# Autodesk Inventor assembly: ASY MSC 002 отстойник осветлитель
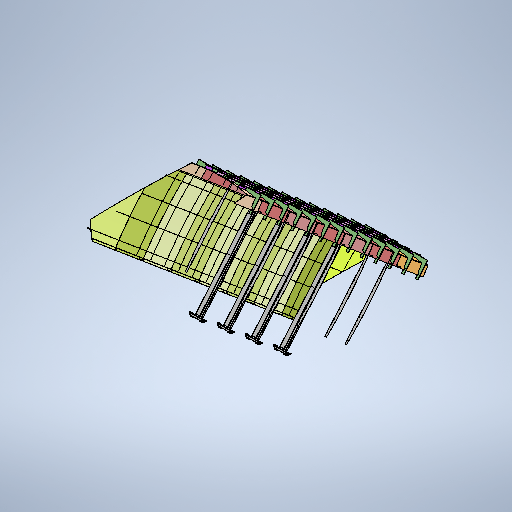
[picture p0: Inventor's stored thumbnail of the model, 512x512]
Saved by Autodesk Inventor 2025.1 (Build 291241020, 241B)
## iProperties
allow_slope_adjustment: 0 ul
flow_configuration: 1 ul
flow_direction: 2 ul
loss_method: 0 ul
radius: 110.000 mm
flow_configuration2: 1 ul
radius: 61.000 mm
radius: 44.450 mm
radius: 59.000 mm
Created: 2024-09-05
Part Number: ASY MSC 002 отстойник осветлитель
Document SubType Name: Assembly
Designer: admin
Mass: 3.32073e+06 g
Surface Area: 6.08214e+06 cm^2
Volume: 433030 cm^3
Density: 7.66859 g/cm^3
Author: admin
## Documents named in this file (52)
- C:\Users\user\YandexDisk-badmisterfox\домашниий пк\Inventor\Manturovo\Manturovo_Se-clar\ASY MSC 002 отстойник осветлитель.iam
- C:\Users\user\YandexDisk-badmisterfox\домашниий пк\Inventor\Manturovo\Manturovo_Se-clar\ASY MSC 900.1 base frame.iam
- C:\Users\user\YandexDisk-badmisterfox\домашниий пк\Inventor\Manturovo\Manturovo_Se-clar\ASY MSC 100 cone.iam
- C:\Users\user\YandexDisk-badmisterfox\домашниий пк\Inventor\Manturovo\Manturovo_Se-clar\MSC 401 sheet lowerback.ipt
- C:\Users\user\YandexDisk-badmisterfox\домашниий пк\Inventor\Manturovo\Manturovo_Se-clar\MSC 701 face 1.ipt
- C:\Users\user\YandexDisk-badmisterfox\домашниий пк\Inventor\Manturovo\Manturovo_Se-clar\MSC 705 ridge 3.ipt
- C:\Users\user\YandexDisk-badmisterfox\домашниий пк\Inventor\Manturovo\Manturovo_Se-clar\MSC 713 tube.ipt
- C:\Users\user\YandexDisk-badmisterfox\домашниий пк\Inventor\Manturovo\Manturovo_Se-clar\ISO 5251 Bends 3D without straight ends(90 deg) DN150 11 11.ipt
- C:\Users\user\YandexDisk-badmisterfox\домашниий пк\Inventor\Manturovo\Manturovo_Se-clar\MSC 408 stringer lowerback.ipt
- C:\Users\user\YandexDisk-badmisterfox\домашниий пк\Inventor\Manturovo\Manturovo_Se-clar\MSC 703 face 2.ipt
- C:\Users\user\YandexDisk-badmisterfox\домашниий пк\Inventor\Manturovo\Manturovo_Se-clar\MSC 702 face 3.ipt
- C:\Users\user\YandexDisk-badmisterfox\домашниий пк\Inventor\Manturovo\Manturovo_Se-clar\MSC 704 face 4.ipt
- C:\Users\user\YandexDisk-badmisterfox\домашниий пк\Inventor\Manturovo\Manturovo_Se-clar\ASY MSC 900.3 base frame.iam
- C:\Users\user\YandexDisk-badmisterfox\домашниий пк\Inventor\Manturovo\Manturovo_Se-clar\Pillars\ASY MSC 900.5 base frame.iam
- C:\Users\user\YandexDisk-badmisterfox\домашниий пк\Inventor\Manturovo\Manturovo_Se-clar\Pillars\ASY MSC 900.4  base frame.iam
- C:\Users\user\YandexDisk-badmisterfox\домашниий пк\Inventor\Manturovo\Manturovo_Se-clar\Pillars\ASY MSC 900.6 base frame.iam
- C:\Users\user\YandexDisk-badmisterfox\домашниий пк\Inventor\Manturovo\Manturovo_Se-clar\ASY MSC 200 BACK.iam
- C:\Users\user\YandexDisk-badmisterfox\домашниий пк\Inventor\Manturovo\Manturovo_Se-clar\ASY MSC 300.2 LEFT BOARD.iam
- C:\Users\user\YandexDisk-badmisterfox\домашниий пк\Inventor\Manturovo\Manturovo_Se-clar\ASY MSC 300.1 RIGHT BOARD.iam
- C:\Users\user\YandexDisk-badmisterfox\домашниий пк\Inventor\Manturovo\Manturovo_Se-clar\ASY MSC 500 BELLY.iam
- C:\Users\user\YandexDisk-badmisterfox\домашниий пк\Inventor\Manturovo\Manturovo_Se-clar\ASY MSC 900.2 support.iam
- C:\Users\user\YandexDisk-badmisterfox\домашниий пк\Inventor\Manturovo\Manturovo_Se-clar\ASY MSC 600 cone exit back.iam
- C:\Users\user\YandexDisk-badmisterfox\домашниий пк\Inventor\Manturovo\Manturovo_Se-clar\ASY MSC 800 gills.iam
- C:\Users\user\YandexDisk-badmisterfox\домашниий пк\Inventor\Manturovo\Manturovo_Se-clar\ASY MSC 400 Accsess hatch.iam
- C:\Users\user\YandexDisk-badmisterfox\домашниий пк\Inventor\Manturovo\Manturovo_Se-clar\MSC DIM 000 settler-clarifier.ipt
- C:\Users\user\YandexDisk-badmisterfox\домашниий пк\Inventor\Manturovo\Manturovo_Se-clar\MSC DIM 001 frame.ipt
- C:\Users\user\YandexDisk-badmisterfox\домашниий пк\Inventor\Manturovo\Manturovo_Se-clar\ASY MSC 900.7 base frame transverse.iam
- C:\Users\user\YandexDisk-badmisterfox\домашниий пк\Inventor\Manturovo\Manturovo_Se-clar\ASY MSC 900.8 base frame transverse.iam
- C:\Users\user\YandexDisk-badmisterfox\домашниий пк\Inventor\Manturovo\Manturovo_Se-clar\MSC 908 transverse pillar plate.ipt
- C:\Users\user\YandexDisk-badmisterfox\домашниий пк\Inventor\Manturovo\Manturovo_Se-clar\MSC 900.9 base frame transverse.ipt
- C:\Users\user\YandexDisk-badmisterfox\домашниий пк\Inventor\Manturovo\Manturovo_Se-clar\ASY MSC 700 water tray.iam
- C:\Users\user\YandexDisk-badmisterfox\домашниий пк\Inventor\Manturovo\Manturovo_Se-clar\ASY 940 linkage.iam
- C:\Users\user\YandexDisk-badmisterfox\домашниий пк\Inventor\Manturovo\Manturovo_Se-clar\MSC 510 BELLY PILLAR.ipt
- C:\Users\user\YandexDisk-badmisterfox\домашниий пк\Inventor\Manturovo\Manturovo_Se-clar\ASY MSC 900.7 support.iam
- C:\Users\user\YandexDisk-badmisterfox\домашниий пк\Inventor\Manturovo\Manturovo_Se-clar\Content Center Files\en-US\DIN 2605 90 T 3\DIN 2605 90 Deg Elbow Type 2 168.3 - 2.6S.ipt
- C:\Users\admin\YandexDisk-badmisterfox\домашниий пк\Inventor\Manturovo\Manturovo_Se-clar\3d party\Stamp flange DIN2642\Stamd flange lapped collar DIN2642.ipt
- C:\Users\user\YandexDisk-badmisterfox\домашниий пк\Inventor\Manturovo\Manturovo_Se-clar\3d party\Stamp flange DIN2642\Stamd flange lapped collar DIN2642\Stamp flange DIN2642-150.ipt
- C:\Users\user\YandexDisk-badmisterfox\домашниий пк\Inventor\Manturovo\Manturovo_Se-clar\Content Center Files\en-US\DIN 2605 90 T 3\DIN 2605 90 Deg Elbow Type 2 88.9 - 2.3S.ipt
- C:\Users\user\YandexDisk-badmisterfox\домашниий пк\Inventor\Manturovo\Manturovo_Se-clar\Stamp flange DIN2642-080.ipt
- C:\Users\user\YandexDisk-badmisterfox\домашниий пк\Inventor\Manturovo\Manturovo_Se-clar\DIN EN ISO 1127(1) - 88,9 x 2,3 - 100.ipt
- C:\Users\user\YandexDisk-badmisterfox\домашниий пк\Inventor\Manturovo\Manturovo_Se-clar\3d party\Stamp flange DIN2642\Stamd flange lapped collar DIN2642.ipt
- C:\Users\user\YandexDisk-badmisterfox\домашниий пк\Inventor\Manturovo\Manturovo_Se-clar\3d party\Butterfly value\butterfly-valve-3-in-1.snapshot.4\vpe_3449-02_dn80_.iam
- C:\Users\user\YandexDisk-badmisterfox\домашниий пк\Inventor\Manturovo\Manturovo_Se-clar\LASER\4 очередь\D-ring 11.ipt
- C:\Users\user\YandexDisk-badmisterfox\домашниий пк\Inventor\Manturovo\Manturovo_Se-clar\MSC 606 rocket tube 6.ipt
- C:\Users\user\YandexDisk-badmisterfox\домашниий пк\Inventor\Manturovo\Manturovo_Se-clar\Stamp flange DIN2642-065.ipt
- C:\Users\user\YandexDisk-badmisterfox\домашниий пк\Inventor\Manturovo\Manturovo_Se-clar\ContentCenter\en-US\ISO 5251 B 3D\ISO 5251 Bends 3D without straight ends(90 deg) DN65 2.9 2.9.ipt
- C:\Users\user\YandexDisk-badmisterfox\домашниий пк\Inventor\Manturovo\Manturovo_Se-clar\MSC 616 belly tube 16.ipt
- C:\Users\user\YandexDisk-badmisterfox\домашниий пк\Inventor\Manturovo\Manturovo_Se-clar\MSC 617 belly tube 17.ipt
- C:\Users\user\YandexDisk-badmisterfox\домашниий пк\Inventor\Manturovo\Manturovo_Se-clar\MSC 618 belly tube 18.ipt
- C:\Users\user\YandexDisk-badmisterfox\домашниий пк\Inventor\Manturovo\Manturovo_Se-clar\MSC 808 sheet.ipt
- C:\Users\user\YandexDisk-badmisterfox\домашниий пк\Inventor\Manturovo\Manturovo_Se-clar\DIN EN 10219-2 - 40 x 20 x 2  - 2000.ipt
- C:\Users\user\YandexDisk-badmisterfox\домашниий пк\Inventor\Manturovo\Manturovo_Se-clar\MSC 813 wall support gills.ipt
## Components (80 placed, 52 different names)
1. MSC DIM 000 settler-clarifier.ipt:1
2. MSC DIM 001 frame.ipt:1
3. ASY MSC 900.4  base frame.iam:1 [sub-assembly] — Mate:32, Mate:33, Mate:45, Mate:46, Cylindrical:11, Mate:82
4. ASY MSC 900.5 base frame.iam:1 [sub-assembly] — Flush:11, Cylindrical:7, Mate:46, Mate:48, Cylindrical:10
5. ASY MSC 900.6 base frame.iam:1 [sub-assembly] — Mate:38, Mate:39, Cylindrical:6, Mate:47, Rigid:19, Rigid:20, Rigid:21, Rigid:22, Cylindrical:9, Mate:84
6. ASY MSC 900.3 base frame.iam:1 [sub-assembly] — Mate:23, Mate:24, Mate:44, Mate:45, Rigid:31, Rigid:32, Rigid:33, Cylindrical:8
7. ASY MSC 900.8 base frame transverse.iam:1 [sub-assembly] — Rigid:22
8. ASY MSC 900.8 base frame transverse.iam:2 [sub-assembly] — Rigid:21
9. ASY MSC 900.7 base frame transverse.iam:1 [sub-assembly] — Rigid:19
10. ASY MSC 900.7 base frame transverse.iam:2 [sub-assembly] — Rigid:20
11. MSC 705 ridge 3.ipt:1
12. MSC 704 face 4.ipt:1
13. MSC 900.9 base frame transverse.ipt:4 — Mate:81, Mate:83
14. Part1:2 — Mate:81, Mate:82
15. Part1:4 — Mate:88
16. MSC 900.9 base frame transverse:7 — Mate:87, Mate:88
17. ASY MSC 900.2 support.iam:5 [sub-assembly]
18. ASY MSC 900.7 support:2 [sub-assembly] — Cylindrical:11, Mate:78
19. Part1:3 — Mate:84, Mate:85
20. MSC 900.9 base frame transverse.ipt:1 — Mate:85, Mate:86
21. MSC 900.9 base frame transverse.ipt:2
22. ASY MSC 900.2 support.iam:4 [sub-assembly] — Cylindrical:7, Mate:41
23. ASY MSC 900.7 support:3 [sub-assembly] — Cylindrical:10, Mate:79
24. MSC 701 face 1.ipt:1 — Rigid:4, Flush:9, Mate:35, Rigid:35, Rigid:36, Rigid:39, Rigid:40
25. ASY MSC 900.2 support.iam:1 [sub-assembly] — Cylindrical:6, Mate:42
26. MSC 702 face 3.ipt:1 — Mate:34, Mate:35, Mate:36, Mate:66
27. MSC 703 face 2.ipt:1 — Flush:13, Flush:17, Mate:66
28. MSC 713 tube.ipt:2
29. ISO 5251 Bends 3D without straight ends(90 deg) DN150 11 11.ipt:1
30. MSC 713 tube.ipt:1 — Rigid:4
31. ASY MSC 900.7 support:4 [sub-assembly] — Cylindrical:9, Mate:80
32. ASY MSC 700 water tray.iam:1 [sub-assembly]
33. Part1.ipt:1 — Rigid:33, Mate:68, Mate:69, Mate:70
34. MSC 900.9 base frame transverse.ipt:3 — Mate:68, Mate:69, Mate:70
35. ASY MSC 900.2 support.iam:8 [sub-assembly]
36. ASY MSC 900.7 support:1 [sub-assembly] — Cylindrical:8, Mate:77
37. ASY MSC 600 cone exit back.iam:1 [sub-assembly] — Rigid:17
38. MSC 908 transverse pillar plate.ipt:1
39. MSC 908 transverse pillar plate.ipt:2 — Mate:50, Flush:16, Flush:18
40. MSC 401 sheet lowerback.ipt:1 — Mate:29, Mate:30, Rigid:34
41. ASY MSC 400 Accsess hatch.iam:1 [sub-assembly] — Rigid:34
42. MSC 408 stringer lowerback.ipt:2
43. MSC 408 stringer lowerback.ipt:1
44. ASY MSC 100 cone.iam:1 [sub-assembly] — Mate:19, Flush:6, Mate:29, Rigid:17, Rigid:48, Rigid:53
45. ASY MSC 900.1 base frame.iam:1 [sub-assembly] — Flush:5, Mate:19, Mate:44, Mate:47, Mate:50, Flush:16
46. ASY 940 linkage.iam:1 [sub-assembly] — Rigid:32, Flush:18
47. ASY 940 linkage.iam:2 [sub-assembly] — Rigid:31
48. ASY MSC 500 BELLY.iam:1 [sub-assembly] — Flush:7, Mate:22, Rigid:10, Rigid:11, Mate:41, Mate:42, Mate:77, Mate:78, Mate:79, Mate:80, Mate:83, Mate:86, Mate:87
49. ASY MSC 200 BACK.iam:1 [sub-assembly] — Flush:8
50. ASY MSC 300.2 LEFT BOARD.iam:1 [sub-assembly] — Rigid:11, Mate:34, Rigid:49
51. ASY MSC 300.1 RIGHT BOARD.iam:1 [sub-assembly] — Rigid:10, Flush:17
52. ASY MSC 800 gills.iam:1 [sub-assembly] — Mate:22, Rigid:56
53. DIN 2605 90 Deg Elbow Type 2 168.3 - 2.6S:1 — Rigid:36, Rigid:38
54. DIN 2605 90 Deg Elbow Type 2 168.3 - 2.6S:2 — Rigid:35, Rigid:37
55. Stamp flange DIN2642-150:1 — Rigid:38
56. Stamp flange DIN2642-150:3 — Rigid:37
57. DIN 2605 90 Deg Elbow Type 2 88.9 - 2.3S:1 — Rigid:39, Rotational:2
58. Stamp flange DIN2642-080:4 — Rotational:2
59. DIN EN ISO 1127(1) - 88,9 x 2,3 - 100:1 — Rigid:40
60. vpe_3449-02_dn80_:1 [sub-assembly] — Rigid:48
61. D-ring 11:1 — Rigid:41, Rigid:49
62. D-ring 11:2 — Rigid:41
63. MSC 606 rocket tube 6.ipt:1 — Rotational:4
64. ISO 5251 Bends 3D without straight ends(90 deg) DN65 2.9:1 — Rigid:45, Rigid:47
65. Stamp flange DIN2642-065.ipt:1 — Rotational:3, Rotational:6
66. ISO 5251 Bends 3D without straight ends(90 deg) DN65 2.9:2 — Rotational:3, Rigid:46
67. MSC 616 belly tube 16:1 — Rigid:45, Rigid:46
68. Stamp flange DIN2642-065:6 — Rigid:47, Rotational:5
69. Stamp flange DIN2642-065:7 — Rotational:4, Rotational:5
70. Stamp flange DIN2642-065:8 — Rotational:6, Rotational:7
71. MSC 617 belly tube 17:1 — Rotational:7, Rigid:50
72. Stamp flange DIN2642-065:9 — Rigid:50, Rigid:55
73. MSC 618 belly tube 18:1 — Rigid:52, Rigid:51
74. Stamp flange DIN2642-065:10 — Rigid:53, Rigid:52
75. Stamp flange DIN2642-065:11 — Rigid:51, Rigid:54
76. vpe_3449-02_dn80_:2 [sub-assembly] — Rigid:54
77. vpe_3449-02_dn80_:3 [sub-assembly] — Rigid:55
78. MSC 808 sheet:1
79. DIN EN 10219-2 - 40 x 20 x 2  - 2000:1
80. MSC 813 wall support gills:1 — Rigid:56
## Relationships (111: Mate 47, WeldJoint 37, Flush 12, CylindricalJoint 8, RevoluteJoint 7)
- [Mate]: MSC 401 sheet lowerback.ipt:1 ↔ ASY MSC 100 cone.iam:1
- [WeldJoint]: ISO 5251 Bends 3D without straight ends(90 deg) DN150 11 11.ipt:1 ↔ MSC 713 tube.ipt:1
- [Mate]: MSC 408 stringer lowerback.ipt:1 ↔ ASY MSC 100 cone.iam:1
- [RevoluteJoint]: MSC 713 tube.ipt:2 ↔ ISO 5251 Bends 3D without straight ends(90 deg) DN150 11 11.ipt:1
- Rigid:4 [WeldJoint]: MSC 701 face 1.ipt:1 ↔ MSC 713 tube.ipt:1
- [Mate]: MSC 408 stringer lowerback.ipt:2 ↔ ASY MSC 100 cone.iam:1
- [Mate]: ASY MSC 600 cone exit back.iam:1 ↔ ASY MSC 500 BELLY.iam:1
- [WeldJoint]: MSC 705 ridge 3.ipt:1 ↔ ASY MSC 700 water tray.iam:1
- [WeldJoint]: MSC 705 ridge 3.ipt:1 ↔ ASY MSC 700 water tray.iam:1
- [Flush]: ASY MSC 600 cone exit back.iam:1 ↔ ASY MSC 500 BELLY.iam:1
- [Mate]: ASY MSC 500 BELLY.iam:1 ↔ ASY MSC 800 gills.iam:1
- [Mate]: MSC 701 face 1.ipt:1 ↔ ASY MSC 500 BELLY.iam:1
- [Mate] (3 mm): MSC 701 face 1.ipt:1 ↔ ASY MSC 500 BELLY.iam:1
- [Mate] (3 mm): ASY MSC 900.2 support.iam:5 ↔ ASY MSC 500 BELLY.iam:1
- [Mate] (3 mm): ASY MSC 900.2 support.iam:8 ↔ ASY MSC 500 BELLY.iam:1
- [CylindricalJoint]: ASY MSC 900.4  base frame.iam:1 ↔ ASY MSC 900.2 support.iam:5
- [Mate] (-2860 mm): ASY MSC 500 BELLY.iam:1 ↔ ASY MSC 200 BACK.iam:1
- [CylindricalJoint]: ASY MSC 900.3 base frame.iam:1 ↔ ASY MSC 900.2 support.iam:8
- [Flush]: ASY MSC 900.4  base frame.iam:1 ↔ ASY MSC 900.3 base frame.iam:1
- Flush:5: ASY MSC 900.1 base frame.iam:1
- Mate:19: ASY MSC 100 cone.iam:1 ↔ ASY MSC 900.1 base frame.iam:1
- Flush:6: ASY MSC 100 cone.iam:1
- Flush:7: ASY MSC 500 BELLY.iam:1
- Flush:8: ASY MSC 200 BACK.iam:1
- Mate:22: ASY MSC 500 BELLY.iam:1 ↔ ASY MSC 800 gills.iam:1
- Mate:23: ASY MSC 900.3 base frame.iam:1
- Mate:24: ASY MSC 900.3 base frame.iam:1
- Flush:9: MSC 701 face 1.ipt:1
- Mate:29: MSC 401 sheet lowerback.ipt:1 ↔ ASY MSC 100 cone.iam:1
- Mate:30: MSC 401 sheet lowerback.ipt:1
- Rigid:10 [WeldJoint] (-25 mm): ASY MSC 500 BELLY.iam:1 ↔ ASY MSC 300.1 RIGHT BOARD.iam:1
- Rigid:11 [WeldJoint] (-25 mm): ASY MSC 500 BELLY.iam:1 ↔ ASY MSC 300.2 LEFT BOARD.iam:1
- Flush:11: ASY MSC 900.5 base frame.iam:1
- Mate:32: ASY MSC 900.4  base frame.iam:1
- Mate:33: ASY MSC 900.4  base frame.iam:1
- Mate:34: MSC 702 face 3.ipt:1 ↔ ASY MSC 300.2 LEFT BOARD.iam:1
- Mate:35: MSC 701 face 1.ipt:1 ↔ MSC 702 face 3.ipt:1
- [WeldJoint]: MSC 705 ridge 3.ipt:1 ↔ ASY MSC 700 water tray.iam:1
- Mate:36: MSC 702 face 3.ipt:1
- Mate:38: ASY MSC 900.6 base frame.iam:1
- Mate:39: ASY MSC 900.6 base frame.iam:1
- Cylindrical:6: ASY MSC 900.6 base frame.iam:1 ↔ ASY MSC 900.2 support.iam:1
- Cylindrical:7: ASY MSC 900.5 base frame.iam:1 ↔ ASY MSC 900.2 support.iam:4
- Mate:41 (3 mm): ASY MSC 900.2 support.iam:4 ↔ ASY MSC 500 BELLY.iam:1
- Mate:42 (3 mm): ASY MSC 900.2 support.iam:1 ↔ ASY MSC 500 BELLY.iam:1
- Flush:13: MSC 703 face 2.ipt:1
- Mate:44 (820 mm): ASY MSC 900.3 base frame.iam:1 ↔ ASY MSC 900.1 base frame.iam:1
- Mate:45 (1430 mm): ASY MSC 900.4  base frame.iam:1 ↔ ASY MSC 900.3 base frame.iam:1
- Mate:46 (1430 mm): ASY MSC 900.4  base frame.iam:1 ↔ ASY MSC 900.5 base frame.iam:1
- Mate:47 (5300 mm): ASY MSC 900.6 base frame.iam:1 ↔ ASY MSC 900.1 base frame.iam:1
- Rigid:17 [WeldJoint]: ASY MSC 600 cone exit back.iam:1 ↔ ASY MSC 100 cone.iam:1
- Mate:48: ASY MSC 900.5 base frame.iam:1
- Rigid:19 [WeldJoint]: ASY MSC 900.6 base frame.iam:1 ↔ ASY MSC 900.7 base frame transverse.iam:1
- Rigid:20 [WeldJoint]: ASY MSC 900.6 base frame.iam:1 ↔ ASY MSC 900.7 base frame transverse.iam:2
- Rigid:21 [WeldJoint]: ASY MSC 900.6 base frame.iam:1 ↔ ASY MSC 900.8 base frame transverse.iam:2
- Rigid:22 [WeldJoint]: ASY MSC 900.6 base frame.iam:1 ↔ ASY MSC 900.8 base frame transverse.iam:1
- Mate:50: MSC 908 transverse pillar plate.ipt:2 ↔ ASY MSC 900.1 base frame.iam:1
- Flush:16 (-40 mm): MSC 908 transverse pillar plate.ipt:2 ↔ ASY MSC 900.1 base frame.iam:1
- Flush:17: MSC 703 face 2.ipt:1 ↔ ASY MSC 300.1 RIGHT BOARD.iam:1
- Mate:66: MSC 702 face 3.ipt:1 ↔ MSC 703 face 2.ipt:1
- [WeldJoint]: MSC 908 transverse pillar plate.ipt:1 ↔ ASY 940 linkage.iam:2
- Rigid:31 [WeldJoint]: ASY MSC 900.3 base frame.iam:1 ↔ ASY 940 linkage.iam:2
- Rigid:32 [WeldJoint]: ASY MSC 900.3 base frame.iam:1 ↔ ASY 940 linkage.iam:1
- Flush:18: MSC 908 transverse pillar plate.ipt:2 ↔ ASY 940 linkage.iam:1
- Rigid:33 [WeldJoint]: ASY MSC 900.3 base frame.iam:1 ↔ Part1.ipt:1
- Mate:68: Part1.ipt:1 ↔ MSC 900.9 base frame transverse.ipt:3
- Mate:69 (11 mm): Part1.ipt:1 ↔ MSC 900.9 base frame transverse.ipt:3
- Mate:70: Part1.ipt:1 ↔ MSC 900.9 base frame transverse.ipt:3
- Cylindrical:8: ASY MSC 900.3 base frame.iam:1 ↔ ASY MSC 900.7 support:1
- Mate:77: ASY MSC 900.7 support:1 ↔ ASY MSC 500 BELLY.iam:1
- Cylindrical:9: ASY MSC 900.6 base frame.iam:1 ↔ ASY MSC 900.7 support:4
- Cylindrical:10: ASY MSC 900.5 base frame.iam:1 ↔ ASY MSC 900.7 support:3
- Cylindrical:11: ASY MSC 900.4  base frame.iam:1 ↔ ASY MSC 900.7 support:2
- Mate:78: ASY MSC 900.7 support:2 ↔ ASY MSC 500 BELLY.iam:1
- Mate:79: ASY MSC 900.7 support:3 ↔ ASY MSC 500 BELLY.iam:1
- Mate:80: ASY MSC 900.7 support:4 ↔ ASY MSC 500 BELLY.iam:1
- Mate:81: MSC 900.9 base frame transverse.ipt:4 ↔ Part1:2
- Mate:82: ASY MSC 900.4  base frame.iam:1 ↔ Part1:2
- Mate:83: MSC 900.9 base frame transverse.ipt:4 ↔ ASY MSC 500 BELLY.iam:1
- Mate:84: ASY MSC 900.6 base frame.iam:1 ↔ Part1:3
- Mate:85: Part1:3 ↔ MSC 900.9 base frame transverse.ipt:1
- Mate:86: MSC 900.9 base frame transverse.ipt:1 ↔ ASY MSC 500 BELLY.iam:1
- Mate:87: MSC 900.9 base frame transverse:7 ↔ ASY MSC 500 BELLY.iam:1
- Mate:88: Part1:4 ↔ MSC 900.9 base frame transverse:7
- Rigid:34 [WeldJoint]: MSC 401 sheet lowerback.ipt:1 ↔ ASY MSC 400 Accsess hatch.iam:1
- Rigid:35 [WeldJoint]: MSC 701 face 1.ipt:1 ↔ DIN 2605 90 Deg Elbow Type 2 168.3 - 2.6S:2
- Rigid:36 [WeldJoint]: MSC 701 face 1.ipt:1 ↔ DIN 2605 90 Deg Elbow Type 2 168.3 - 2.6S:1
- Rigid:37 [WeldJoint]: DIN 2605 90 Deg Elbow Type 2 168.3 - 2.6S:2 ↔ Stamp flange DIN2642-150:3
- Rigid:38 [WeldJoint]: DIN 2605 90 Deg Elbow Type 2 168.3 - 2.6S:1 ↔ Stamp flange DIN2642-150:1
- Rigid:39 [WeldJoint] (-100 mm): MSC 701 face 1.ipt:1 ↔ DIN 2605 90 Deg Elbow Type 2 88.9 - 2.3S:1
- Rotational:2 [RevoluteJoint]: DIN 2605 90 Deg Elbow Type 2 88.9 - 2.3S:1 ↔ Stamp flange DIN2642-080:4
- Rigid:40 [WeldJoint]: MSC 701 face 1.ipt:1 ↔ DIN EN ISO 1127(1) - 88,9 x 2,3 - 100:1
- Rigid:41 [WeldJoint]: D-ring 11:1 ↔ D-ring 11:2
- [WeldJoint]: ASY MSC 600 cone exit back.iam:1 ↔ MSC 606 rocket tube 6.ipt:1
- Rotational:3 [RevoluteJoint]: Stamp flange DIN2642-065.ipt:1 ↔ ISO 5251 Bends 3D without straight ends(90 deg) DN65 2.9:2
- Rigid:45 [WeldJoint]: ISO 5251 Bends 3D without straight ends(90 deg) DN65 2.9:1 ↔ MSC 616 belly tube 16:1
- Rigid:46 [WeldJoint]: ISO 5251 Bends 3D without straight ends(90 deg) DN65 2.9:2 ↔ MSC 616 belly tube 16:1
- Rigid:47 [WeldJoint]: ISO 5251 Bends 3D without straight ends(90 deg) DN65 2.9:1 ↔ Stamp flange DIN2642-065:6
- Rotational:4 [RevoluteJoint]: MSC 606 rocket tube 6.ipt:1 ↔ Stamp flange DIN2642-065:7
- Rotational:5 [RevoluteJoint]: Stamp flange DIN2642-065:6 ↔ Stamp flange DIN2642-065:7
- Rotational:6 [RevoluteJoint]: Stamp flange DIN2642-065.ipt:1 ↔ Stamp flange DIN2642-065:8
- Rigid:48 [WeldJoint]: ASY MSC 100 cone.iam:1 ↔ vpe_3449-02_dn80_:1
- Rigid:49 [WeldJoint]: ASY MSC 300.2 LEFT BOARD.iam:1 ↔ D-ring 11:1
- Rotational:7 [RevoluteJoint]: Stamp flange DIN2642-065:8 ↔ MSC 617 belly tube 17:1
- Rigid:50 [WeldJoint]: MSC 617 belly tube 17:1 ↔ Stamp flange DIN2642-065:9
- Rigid:53 [WeldJoint]: ASY MSC 100 cone.iam:1 ↔ Stamp flange DIN2642-065:10
- Rigid:52 [WeldJoint]: MSC 618 belly tube 18:1 ↔ Stamp flange DIN2642-065:10
- Rigid:51 [WeldJoint]: MSC 618 belly tube 18:1 ↔ Stamp flange DIN2642-065:11
- Rigid:54 [WeldJoint]: Stamp flange DIN2642-065:11 ↔ vpe_3449-02_dn80_:2
- Rigid:55 [WeldJoint]: Stamp flange DIN2642-065:9 ↔ vpe_3449-02_dn80_:3
- Rigid:56 [WeldJoint] (700 mm): ASY MSC 800 gills.iam:1 ↔ MSC 813 wall support gills:1
## Named parameters: d334_d122 = 0 mm
